# Autodesk Inventor assembly: EE_base_assembly
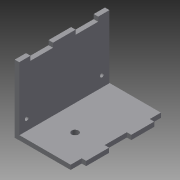
[picture p0: Inventor's stored thumbnail of the model, 180x180]
Saved by Autodesk Inventor 2015 (Build 190159000, 159)
## iProperties
Created: 2017-03-04
Part Number: EE_base_assembly
Document SubType Name: Assembly
Designer: Guy
Author: Guy
## Documents named in this file (4)
- C:\Users\Ernest\Documents\Capstone-Project\doc\CAD\LowLevel_Rev3\EE_base\EE_base_assembly.iam
- C:\Users\Ernest\Documents\Capstone-Project\doc\CAD\LowLevel_Rev3\EE_base\bottom.ipt
- C:\Users\Ernest\Documents\Capstone-Project\doc\CAD\LowLevel_Rev3\EE_base\Side.ipt
- C:\Users\Ernest\Documents\Capstone-Project\doc\CAD\LowLevel_Rev3\EE_base\top.ipt
## Components (4 placed, 3 different names)
1. bottom:1 — Mate:3, Flush:3, Flush:4
2. Side:1 — Flush:1, Mate:1, Mate:2, Mate:3, Flush:3, Flush:4
3. Side:2 — Flush:2, Flush:5, Mate:4
4. top:1 — Flush:1, Mate:1, Mate:2, Flush:2, Flush:5, Mate:4
## Relationships (9: Flush 5, Mate 4)
- Flush:1: Side:1 ↔ top:1
- Mate:1: Side:1 ↔ top:1
- Mate:2: Side:1 ↔ top:1
- Flush:2: Side:2 ↔ top:1
- Mate:3: bottom:1 ↔ Side:1
- Flush:3: bottom:1 ↔ Side:1
- Flush:4: bottom:1 ↔ Side:1
- Flush:5: Side:2 ↔ top:1
- Mate:4: Side:2 ↔ top:1
